# Autodesk Inventor assembly: Assembly no buttons
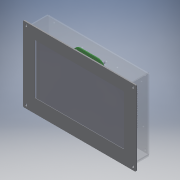
[picture p0: Inventor's stored thumbnail of the model, 180x180]
Saved by Autodesk Inventor 2019 (Build 230136000, 136)
## iProperties
Created: 2021-10-03
Part Number: Assembly no buttons
Document SubType Name: Assembly
Designer: maxwe
Author: maxwe
## Documents named in this file (5)
- D:\Makerplane_Efis\EFIS-Hardware-7-inch\New Enclosure\Assembly no buttons.iam
- D:\Makerplane_Efis\EFIS-Hardware-7-inch\New Enclosure\Front Panel no buttons.iam
- D:\Makerplane_Efis\EFIS-Hardware-7-inch\New Enclosure\NHD-7.ipt
- D:\Makerplane_Efis\EFIS-Hardware-7-inch\New Enclosure\CapeBeagleBoneCape.ipt
- D:\Makerplane_Efis\EFIS-Hardware-7-inch\New Enclosure\Back Case No Buttons.ipt
## Components (4 placed, 4 different names)
1. Front Panel no buttons:1 [sub-assembly] — Cylindrical:1, Mate:1, Angle:1, Cylindrical:2, Mate:5, Angle:2
2. NHD-7:1 — Cylindrical:1, Mate:1, Angle:1, Mate:2, Mate:3, Mate:4
3. CapeBeagleBoneCape:2 — Mate:2, Mate:3, Mate:4
4. Back Case No Buttons:1 — Cylindrical:2, Mate:5, Angle:2
## Relationships (9: Mate 5, CylindricalJoint 2, Angle 2)
- Cylindrical:1: Front Panel no buttons:1 ↔ NHD-7:1
- Mate:1: Front Panel no buttons:1 ↔ NHD-7:1
- Angle:1 (0 deg): Front Panel no buttons:1 ↔ NHD-7:1
- Mate:2: NHD-7:1 ↔ CapeBeagleBoneCape:2
- Mate:3: NHD-7:1 ↔ CapeBeagleBoneCape:2
- Mate:4: NHD-7:1 ↔ CapeBeagleBoneCape:2
- Cylindrical:2: Front Panel no buttons:1 ↔ Back Case No Buttons:1
- Mate:5: Front Panel no buttons:1 ↔ Back Case No Buttons:1
- Angle:2 (0 deg): Front Panel no buttons:1 ↔ Back Case No Buttons:1
